# Autodesk Inventor assembly: Diff_test
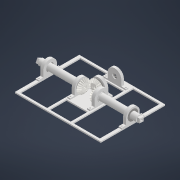
[picture p0: Inventor's stored thumbnail of the model, 180x180]
Saved by Autodesk Inventor 2021 (Build 250183000, 183)
## iProperties
Created: 2021-01-24
Part Number: Diff_test
Document SubType Name: Assembly
Designer: Ctroi
Author: Ctroi
## Documents named in this file (9)
- G:\Roverprojekt\Github Projekt\Rover\Diff_test.iam
- G:\Roverprojekt\Github Projekt\Rover\Testplatte_Differential.ipt
- G:\Roverprojekt\Github Projekt\Rover\Halterung_Differential.ipt
- G:\Roverprojekt\Github Projekt\Rover\Kugellager.ipt
- G:\Roverprojekt\Github Projekt\Rover\Halterung_Differential_2.ipt
- G:\Roverprojekt\Github Projekt\Rover\Verbindung_Rocker_Body.ipt
- G:\Roverprojekt\Github Projekt\Rover\Kegelrad.ipt
- G:\Roverprojekt\Github Projekt\Rover\Halterung_Differential_Mitte.ipt
- G:\Roverprojekt\Github Projekt\Rover\Kugellager_klein.ipt
## Components (18 placed, 8 different names)
1. Testplatte_Differential:1 — Passend:5, Passend:6, Passend:7, Passend:8, Passend:9, Passend:10, Passend:29, Passend:30, Passend:31, Passend:32, Passend:33, Passend:34, Passend:39, Passend:40, Passend:41
2. Kugellager:1 — Passend:37, Passend:38
3. Kugellager:2 — Passend:35, Passend:36
4. Halterung_Differential:1 — Passend:8, Passend:9, Passend:10, Passend:13, Passend:14, Passend:16, Passend:17
5. Halterung_Differential:2 — Passend:5, Passend:6, Passend:7, Passend:11, Passend:12, Passend:15
6. Kugellager:3 — Passend:11, Passend:12, Passend:25, Passend:26
7. Kugellager:4 — Passend:13, Passend:14, Passend:20, Passend:21
8. Halterung_Differential_2:1 — Passend:15, Passend:16, Passend:17, Passend:18, Passend:19
9. Kugellager:5 — Passend:18, Passend:19
10. Verbindung_Rocker_Body:1 — Passend:20, Passend:21, Passend:22, Passend:23, Passend:24
11. Kegelrad2:1 — Passend:22, Passend:23, Passend:24
12. Kegelrad2:2
13. Verbindung_Rocker_Body:2 — Passend:25, Passend:26, Passend:27, Passend:28
14. Kegelrad2:3 — Passend:27, Passend:28
15. Halterung_Differential:3 — Passend:32, Passend:33, Passend:34, Passend:35, Passend:36
16. Halterung_Differential:4 — Passend:29, Passend:30, Passend:31, Passend:37, Passend:38
17. Halterung_Differential_Mitte:1 — Passend:39, Passend:40, Passend:41, Passend:42, Passend:43
18. Kugellager_klein:1 — Passend:42, Passend:43
## Relationships (39: Mate 39)
- Passend:5 [Mate]: Testplatte_Differential:1 ↔ Halterung_Differential:2
- Passend:6 [Mate]: Testplatte_Differential:1 ↔ Halterung_Differential:2
- Passend:7 [Mate]: Testplatte_Differential:1 ↔ Halterung_Differential:2
- Passend:8 [Mate]: Testplatte_Differential:1 ↔ Halterung_Differential:1
- Passend:9 [Mate]: Testplatte_Differential:1 ↔ Halterung_Differential:1
- Passend:10 [Mate]: Testplatte_Differential:1 ↔ Halterung_Differential:1
- Passend:11 [Mate]: Halterung_Differential:2 ↔ Kugellager:3
- Passend:12 [Mate]: Halterung_Differential:2 ↔ Kugellager:3
- Passend:13 [Mate]: Halterung_Differential:1 ↔ Kugellager:4
- Passend:14 [Mate]: Halterung_Differential:1 ↔ Kugellager:4
- Passend:15 [Mate]: Halterung_Differential:2 ↔ Halterung_Differential_2:1
- Passend:16 [Mate]: Halterung_Differential:1 ↔ Halterung_Differential_2:1
- Passend:17 [Mate]: Halterung_Differential:1 ↔ Halterung_Differential_2:1
- Passend:18 [Mate]: Halterung_Differential_2:1 ↔ Kugellager:5
- Passend:19 [Mate]: Halterung_Differential_2:1 ↔ Kugellager:5
- Passend:20 [Mate]: Kugellager:4 ↔ Verbindung_Rocker_Body:1
- Passend:21 [Mate]: Kugellager:4 ↔ Verbindung_Rocker_Body:1
- Passend:22 [Mate]: Verbindung_Rocker_Body:1 ↔ Kegelrad2:1
- Passend:23 [Mate]: Verbindung_Rocker_Body:1 ↔ Kegelrad2:1
- Passend:24 [Mate]: Verbindung_Rocker_Body:1 ↔ Kegelrad2:1
- Passend:25 [Mate]: Kugellager:3 ↔ Verbindung_Rocker_Body:2
- Passend:26 [Mate]: Kugellager:3 ↔ Verbindung_Rocker_Body:2
- Passend:27 [Mate]: Verbindung_Rocker_Body:2 ↔ Kegelrad2:3
- Passend:28 [Mate]: Verbindung_Rocker_Body:2 ↔ Kegelrad2:3
- Passend:29 [Mate]: Testplatte_Differential:1 ↔ Halterung_Differential:4
- Passend:30 [Mate]: Testplatte_Differential:1 ↔ Halterung_Differential:4
- Passend:31 [Mate]: Testplatte_Differential:1 ↔ Halterung_Differential:4
- Passend:32 [Mate]: Testplatte_Differential:1 ↔ Halterung_Differential:3
- Passend:33 [Mate]: Testplatte_Differential:1 ↔ Halterung_Differential:3
- Passend:34 [Mate]: Testplatte_Differential:1 ↔ Halterung_Differential:3
- Passend:35 [Mate]: Kugellager:2 ↔ Halterung_Differential:3
- Passend:36 [Mate]: Kugellager:2 ↔ Halterung_Differential:3
- Passend:37 [Mate]: Kugellager:1 ↔ Halterung_Differential:4
- Passend:38 [Mate]: Kugellager:1 ↔ Halterung_Differential:4
- Passend:39 [Mate]: Testplatte_Differential:1 ↔ Halterung_Differential_Mitte:1
- Passend:40 [Mate]: Testplatte_Differential:1 ↔ Halterung_Differential_Mitte:1
- Passend:41 [Mate]: Testplatte_Differential:1 ↔ Halterung_Differential_Mitte:1
- Passend:42 [Mate]: Halterung_Differential_Mitte:1 ↔ Kugellager_klein:1
- Passend:43 [Mate]: Halterung_Differential_Mitte:1 ↔ Kugellager_klein:1
